# Autodesk Inventor assembly: inside-join-no-hole
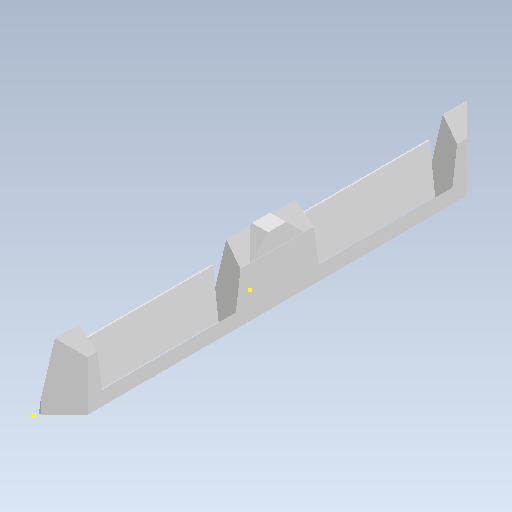
[picture p0: Inventor's stored thumbnail of the model, 512x512]
Saved by Autodesk Inventor 2021 (Build 250183000, 183)
## iProperties
Created: 2020-12-10
Part Number: inside-join-no-hole
Document SubType Name: Assembly
Designer: Luke Kamols
Author: Luke Kamols
## Documents named in this file (3)
- C:\Users\Luke Kamols\OneDrive\Documents\Other\Chess\inside-join-no-hole.iam
- C:\Users\Luke Kamols\OneDrive\Documents\Other\Chess\inside-join-half.ipt
- C:\Users\Luke Kamols\OneDrive\Documents\Other\Chess\middle-join-inside.ipt
## Components (3 placed, 2 different names)
1. inside-join-half:1 — Mate:1, Flush:1, Flush:2, Flush:3, Flush:5
2. inside-join-half:2 — Mate:1, Flush:1, Flush:2, Flush:4
3. middle-join-inside:1 — Flush:3, Flush:4, Flush:5
## Relationships (6: Flush 5, Mate 1)
- Mate:1: inside-join-half:1 ↔ inside-join-half:2
- Flush:1: inside-join-half:1 ↔ inside-join-half:2
- Flush:2: inside-join-half:1 ↔ inside-join-half:2
- Flush:3: inside-join-half:1 ↔ middle-join-inside:1
- Flush:4: inside-join-half:2 ↔ middle-join-inside:1
- Flush:5 (6 mm): inside-join-half:1 ↔ middle-join-inside:1
